# Autodesk Inventor assembly: s-assy-link2
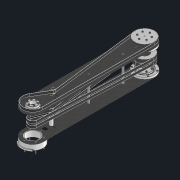
[picture p0: Inventor's stored thumbnail of the model, 180x180]
Saved by Autodesk Inventor 2021 (Build 250183000, 183)
## iProperties
Created: 2021-07-17
Part Number: s-assy-link2
Document SubType Name: Assembly
Designer: yuta0
Mass: 1448.61 g
Surface Area: 6046.34 cm^2
Volume: 815.942 cm^3
Density: 1.77539 g/cm^3
Author: yuta0
## Documents named in this file (23)
- C:\Users\yuta0\Desktop\catchrobo_robot\s-assy-link2.iam
- C:\Users\yuta0\Desktop\catchrobo_robot\carbon_plate3.ipt
- C:\Users\yuta0\Desktop\catchrobo_robot\base30.ipt
- C:\Users\yuta0\Desktop\catchrobo_robot\carbon_plate2.ipt
- C:\Users\yuta0\Desktop\catchrobo_robot\s-assy-link2-bearing.iam
- C:\Users\yuta0\Desktop\catchrobo_robot\s-assy-pulley-j3.iam
- C:\Users\yuta0\Desktop\catchrobo_robot\base14.ipt
- C:\Users\yuta0\Desktop\catchrobo_robot\base3.ipt
- C:\Users\yuta0\Desktop\catchrobo_robot\CB3-20.ipt
- C:\Users\yuta0\Desktop\catchrobo_robot\belt_1.ipt
- C:\Users\yuta0\Desktop\catchrobo_robot\tentioner1.iam
- C:\Users\yuta0\Desktop\catchrobo_robot\CB4-40.ipt
- C:\Users\yuta0\Desktop\catchrobo_robot\base1.ipt
- C:\Users\yuta0\Desktop\catchrobo_robot\belt_2.ipt
- C:\Users\yuta0\Desktop\catchrobo_robot\CC-0814-05.ipt
- C:\Users\yuta0\Desktop\catchrobo_robot\LBNR3.ipt
- C:\Users\yuta0\Desktop\catchrobo_robot\CB3-35.ipt
- C:\Users\yuta0\Desktop\catchrobo_robot\s-assy-spacer2.ipt.iam
- C:\Users\yuta0\Desktop\catchrobo_robot\s-assy-spacer4.iam
- C:\Users\yuta0\Desktop\catchrobo_robot\CBSTNR3-16.ipt
- C:\Users\yuta0\Desktop\catchrobo_robot\base18.ipt
- C:\Users\yuta0\Desktop\catchrobo_robot\SFHRW8-98-M4-N4.ipt
- s-assy-spacer2.ipt
## Components (75 placed, 21 different names)
1. carbon_plate3:1 — メイト:2, メイト:3, メイト:23, メイト:155, メイト:157, メイト:169, メイト:170, メイト:259, メイト:277, メイト:278
2. base30:1 — メイト:1, メイト:2, メイト:3
3. carbon_plate2:1 — メイト:21, メイト:26, メイト:158, メイト:173, メイト:174, メイト:235, メイト:264, メイト:273, メイト:274, メイト:275, メイト:276, メイト:280, メイト:281
4. s-assy-link2-bearing:1 [sub-assembly] — メイト:23, メイト:154, メイト:155, メイト:156, メイト:157, メイト:258
5. s-assy-link2-bearing:2 [sub-assembly] — メイト:26, メイト:158, メイト:159, メイト:233, メイト:252, メイト:263
6. s-assy-pulley-j3:1 [sub-assembly] — メイト:77, メイト:78, メイト:80, メイト:186, メイト:217, メイト:288
7. s-assy-pulley-j3:2 [sub-assembly] — メイト:78, メイト:187, メイト:254, メイト:285
8. base14:1 — メイト:77, メイト:159, メイト:183, メイト:232, メイト:252, メイト:261, メイト:267, メイト:270, メイト:271
9. base3:1 — メイト:47, メイト:48, メイト:80, メイト:154, メイト:156, メイト:260, メイト:269, メイト:286, メイト:289, メイト:290
10. base1:1 — メイト:173, メイト:174, メイト:189, メイト:190, メイト:231, メイト:283
11. belt_1:1 — メイト:183, メイト:231, メイト:232, メイト:250
12. belt_2:2 — メイト:187, メイト:190, メイト:279
13. belt_2:1 — メイト:186, メイト:189, メイト:233
14. base34:1 — メイト:217, メイト:254, メイト:292
15. tentioner1:1 [sub-assembly] — メイト:235, メイト:250
16. s-assy-spacer2.ipt:1 [sub-assembly] — メイト:273, メイト:276, メイト:277
17. s-assy-spacer2.ipt:2 [sub-assembly] — メイト:274, メイト:275
18. s-assy-spacer4:1 [sub-assembly] — メイト:278, メイト:279
19. base18:1 — メイト:285, メイト:286, メイト:291
20. base18:2 — メイト:288, メイト:293
21. SFHRW8-98-M4-N4:1 — メイト:289, メイト:290, メイト:291, メイト:292, メイト:293
22. CB4-40:1 — メイト:169, メイト:170
23. CBSTNR3-16:1 — メイト:280, メイト:281, メイト:282
24. LBNR3:35 — メイト:282, メイト:283
25. CB4-40:2
26. CBSTNR3-16:2
27. LBNR3:36
28. CB4-40:3
29. CBSTNR3-16:3
30. LBNR3:37
31. CB4-40:4
32. CBSTNR3-16:4
33. LBNR3:38
34. CB4-40:5
35. CBSTNR3-16:5
36. LBNR3:39
37. CB4-40:6
38. CBSTNR3-16:6
39. LBNR3:40
40. CB3-35:1 — メイト:270, メイト:271, メイト:272
41. LBNR3:7 — メイト:263, メイト:264
42. LBNR3:13 — メイト:267, メイト:272
43. CB3-20:1 — メイト:47, メイト:48, メイト:268
44. LBNR3:1 — メイト:258, メイト:259
45. LBNR3:14 — メイト:268, メイト:269
46. CB3-35:2
47. LBNR3:15
48. LBNR3:16
49. CB3-20:2
50. LBNR3:17
51. LBNR3:18
52. CB3-35:3
53. LBNR3:19
54. LBNR3:20
55. CB3-20:3
56. LBNR3:21
57. LBNR3:22
58. CB3-35:4
59. LBNR3:23
60. LBNR3:24
61. CB3-20:4
62. LBNR3:25
63. LBNR3:26
64. CB3-35:5
65. LBNR3:27
66. LBNR3:28
67. CB3-20:5
68. LBNR3:29
69. LBNR3:30
70. CB3-35:6
71. LBNR3:31
72. LBNR3:32
73. CB3-20:6
74. LBNR3:33
75. LBNR3:34
## Component patterns: (6 elements, first: CB4-40:1 + CBSTNR3-16:1 + LBNR3:35), (6 elements, first: CB3-35:1 + LBNR3:7 + LBNR3:13 + CB3-20:1 + LBNR3:1 + LBNR3:14)
## Relationships (65: Mate 65)
- メイト:1 [Mate]: base30:1
- メイト:2 [Mate]: carbon_plate3:1 ↔ base30:1
- メイト:3 [Mate]: carbon_plate3:1 ↔ base30:1
- メイト:21 [Mate]: carbon_plate2:1
- メイト:23 [Mate]: carbon_plate3:1 ↔ s-assy-link2-bearing:1
- メイト:26 [Mate]: carbon_plate2:1 ↔ s-assy-link2-bearing:2
- メイト:47 [Mate]: base3:1 ↔ CB3-20:1
- メイト:48 [Mate]: base3:1 ↔ CB3-20:1
- メイト:77 [Mate]: s-assy-pulley-j3:1 ↔ base14:1
- メイト:78 [Mate]: s-assy-pulley-j3:1 ↔ s-assy-pulley-j3:2
- メイト:80 [Mate]: s-assy-pulley-j3:1 ↔ base3:1
- メイト:154 [Mate]: s-assy-link2-bearing:1 ↔ base3:1
- メイト:155 [Mate]: carbon_plate3:1 ↔ s-assy-link2-bearing:1
- メイト:156 [Mate]: s-assy-link2-bearing:1 ↔ base3:1
- メイト:157 [Mate]: carbon_plate3:1 ↔ s-assy-link2-bearing:1
- メイト:158 [Mate]: carbon_plate2:1 ↔ s-assy-link2-bearing:2
- メイト:159 [Mate]: s-assy-link2-bearing:2 ↔ base14:1
- メイト:169 [Mate]: carbon_plate3:1 ↔ CB4-40:1
- メイト:170 [Mate]: carbon_plate3:1 ↔ CB4-40:1
- メイト:173 [Mate]: carbon_plate2:1 ↔ base1:1
- メイト:174 [Mate]: carbon_plate2:1 ↔ base1:1
- メイト:183 [Mate] (0.5 mm): base14:1 ↔ belt_1:1
- メイト:186 [Mate] (0.5 mm): s-assy-pulley-j3:1 ↔ belt_2:1
- メイト:187 [Mate] (0.5 mm): s-assy-pulley-j3:2 ↔ belt_2:2
- メイト:189 [Mate]: base1:1 ↔ belt_2:1
- メイト:190 [Mate]: base1:1 ↔ belt_2:2
- メイト:217 [Mate]: s-assy-pulley-j3:1 ↔ base34:1
- メイト:231 [Mate]: base1:1 ↔ belt_1:1
- メイト:232 [Mate]: base14:1 ↔ belt_1:1
- メイト:233 [Mate]: s-assy-link2-bearing:2 ↔ belt_2:1
- メイト:235 [Mate]: carbon_plate2:1 ↔ tentioner1:1
- メイト:250 [Mate]: belt_1:1 ↔ tentioner1:1
- メイト:252 [Mate]: s-assy-link2-bearing:2 ↔ base14:1
- メイト:254 [Mate]: s-assy-pulley-j3:2 ↔ base34:1
- メイト:258 [Mate]: s-assy-link2-bearing:1 ↔ LBNR3:1
- メイト:259 [Mate]: carbon_plate3:1 ↔ LBNR3:1
- メイト:260 [Mate]: base3:1
- メイト:261 [Mate]: base14:1
- メイト:263 [Mate]: s-assy-link2-bearing:2 ↔ LBNR3:7
- メイト:264 [Mate]: carbon_plate2:1 ↔ LBNR3:7
- メイト:267 [Mate] (2 mm): base14:1 ↔ LBNR3:13
- メイト:268 [Mate]: CB3-20:1 ↔ LBNR3:14
- メイト:269 [Mate] (2 mm): base3:1 ↔ LBNR3:14
- メイト:270 [Mate]: base14:1 ↔ CB3-35:1
- メイト:271 [Mate]: base14:1 ↔ CB3-35:1
- メイト:272 [Mate]: CB3-35:1 ↔ LBNR3:13
- メイト:273 [Mate]: carbon_plate2:1 ↔ s-assy-spacer2.ipt:1
- メイト:274 [Mate]: carbon_plate2:1 ↔ s-assy-spacer2.ipt:2
- メイト:275 [Mate]: carbon_plate2:1 ↔ s-assy-spacer2.ipt:2
- メイト:276 [Mate]: carbon_plate2:1 ↔ s-assy-spacer2.ipt:1
- メイト:277 [Mate]: carbon_plate3:1 ↔ s-assy-spacer2.ipt:1
- メイト:278 [Mate]: carbon_plate3:1 ↔ s-assy-spacer4:1
- メイト:279 [Mate]: belt_2:2 ↔ s-assy-spacer4:1
- メイト:280 [Mate]: carbon_plate2:1 ↔ CBSTNR3-16:1
- メイト:281 [Mate]: carbon_plate2:1 ↔ CBSTNR3-16:1
- メイト:282 [Mate]: CBSTNR3-16:1 ↔ LBNR3:35
- メイト:283 [Mate]: base1:1 ↔ LBNR3:35
- メイト:285 [Mate]: s-assy-pulley-j3:2 ↔ base18:1
- メイト:286 [Mate] (2 mm): base3:1 ↔ base18:1
- メイト:288 [Mate]: s-assy-pulley-j3:1 ↔ base18:2
- メイト:289 [Mate]: base3:1 ↔ SFHRW8-98-M4-N4:1
- メイト:290 [Mate]: base3:1 ↔ SFHRW8-98-M4-N4:1
- メイト:291 [Mate]: base18:1 ↔ SFHRW8-98-M4-N4:1
- メイト:292 [Mate]: base34:1 ↔ SFHRW8-98-M4-N4:1
- メイト:293 [Mate]: base18:2 ↔ SFHRW8-98-M4-N4:1
